# Autodesk Inventor assembly: Wechsel_Zahnrad_fuer_Zahnstange
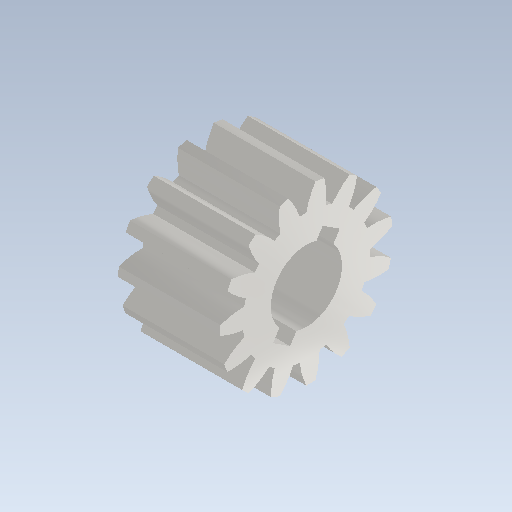
[picture p0: Inventor's stored thumbnail of the model, 512x512]
Saved by Autodesk Inventor 2021 (Build 250183000, 183)
## iProperties
Created: 2021-01-25
Part Number: Wechsel_Zahnrad_fuer_Zahnstange
Document SubType Name: Assembly
Designer: Jaro Machnow
Author: Jaro Machnow
## Documents named in this file (2)
- C:\Users\Jaro Machnow\Documents\Vault\Gruppen\Gruppe 2\Entwurf\Amphibienfahrzeug\Wechsel zwischen Land und Wasser\Mechanik_zum_Wechseln\Wechsel_Zahnrad_fuer_Zahnstange.iam
- C:\Users\Jaro Machnow\Documents\Vault\Gruppen\Gruppe 2\Entwurf\Amphibienfahrzeug\Wechsel zwischen Land und Wasser\Mechanik_zum_Wechseln\Zahnstange\Konstruktions-Assistent\Wechsel_Stirnrad.iam
## Components (1 placed, 1 different names)
1. Stirnräder:2 [sub-assembly] — Passend:1, Passend:2
## Relationships (2: Mate 2)
- Passend:1 [Mate]: Stirnräder:2
- Passend:2 [Mate]: Stirnräder:2
